# Autodesk Inventor assembly: heart
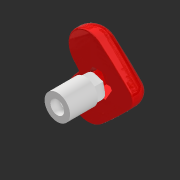
[picture p0: Inventor's stored thumbnail of the model, 180x180]
Saved by Autodesk Inventor 2020.3 (Build 243373010, 373A)
## iProperties
Created: 2021-01-25
Part Number: heart
Document SubType Name: Assembly
Designer: Melvin Strobl
Author: Melvin Strobl
## Documents named in this file (3)
- X:\Heart\heart.iam
- X:\Heart\main.ipt
- X:\Heart\stick.ipt
## Components (2 placed, 2 different names)
1. main:1 — Flush:1, Mate:1
2. stick:1 — Flush:1, Mate:1
## Relationships (2: Flush 1, Mate 1)
- Flush:1 (-15 mm): main:1 ↔ stick:1
- Mate:1: main:1 ↔ stick:1
